# Autodesk Inventor assembly: 垃圾桶底座
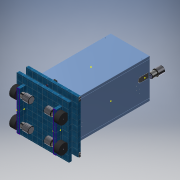
[picture p0: Inventor's stored thumbnail of the model, 180x180]
Saved by Autodesk Inventor 2017 (Build 210142000, 142)
## iProperties
Part Number: 垃圾桶底座
Material: 常规
Document SubType Name: Assembly
Designer: PANDA
Author: PANDA
## Documents named in this file (22)
- D:\PANDA\Study\VG100\P2\草图\垃圾桶丝轴滑杆\垃圾桶底座.iam
- D:\PANDA\Study\VG100\P2\草图\垃圾桶丝轴滑杆\垃圾桶正版.ipt
- D:\PANDA\Study\VG100\P2\草图\垃圾桶丝轴滑杆\垃圾桶侧板.ipt
- D:\PANDA\Study\VG100\P2\草图\垃圾桶丝轴滑杆\垃圾桶底板.ipt
- D:\PANDA\Study\VG100\P2\草图\垃圾桶丝轴滑杆\圆柱.ipt
- D:\PANDA\Study\VG100\P2\草图\垃圾桶丝轴滑杆\马达安装板.ipt
- D:\PANDA\Study\VG100\P2\草图\垃圾桶丝轴滑杆\轮子.ipt
- D:\PANDA\Study\VG100\P2\草图\垃圾桶丝轴滑杆\马达.ipt
- D:\PANDA\Study\VG100\P2\草图\垃圾桶丝轴滑杆\红外.ipt
- D:\PANDA\Study\VG100\P2\草图\垃圾桶丝轴滑杆\红外测距.ipt
- D:\PANDA\Study\VG100\P2\草图\垃圾桶丝轴滑杆\姿态传感器.ipt
- D:\PANDA\Study\VG100\P2\草图\垃圾桶丝轴滑杆\激光传感器.ipt
- D:\PANDA\Study\VG100\P2\草图\垃圾桶丝轴滑杆\内层升降板.ipt
- D:\PANDA\Study\VG100\P2\草图\垃圾桶丝轴滑杆\内层正板.ipt
- D:\PANDA\Study\VG100\P2\草图\垃圾桶丝轴滑杆\内层侧板.ipt
- D:\PANDA\Study\VG100\P2\草图\垃圾桶丝轴滑杆\推杆电机.ipt
- D:\PANDA\Study\VG100\P2\草图\垃圾桶丝轴滑杆\打包支架.ipt
- D:\PANDA\Study\VG100\P2\草图\垃圾桶丝轴滑杆\压缩杆.ipt
- D:\PANDA\Study\VG100\P2\草图\垃圾桶丝轴滑杆\滑竿固定器.ipt
- D:\PANDA\Study\VG100\P2\草图\垃圾桶丝轴滑杆\长轴.ipt
- D:\PANDA\Study\VG100\P2\草图\垃圾桶丝轴滑杆\丝杆.ipt
- D:\PANDA\Study\VG100\P2\草图\垃圾桶丝轴滑杆\升降板.ipt
## Components (59 placed, 21 different names)
1. 垃圾桶正版:1 — 旋转:3, 旋转:7, 旋转:8, 旋转:14
2. 垃圾桶侧板:2 — 旋转:3, 旋转:4, 旋转:5, 旋转:13, 刚性:22, 旋转:67, 旋转:68, 旋转:70, 旋转:81
3. 垃圾桶正版:2 — 旋转:4, 旋转:5, 旋转:6, 旋转:11
4. 垃圾桶侧板:3 — 旋转:6, 旋转:7, 旋转:12, 旋转:58, 旋转:63, 旋转:64, 旋转:65, 旋转:78
5. 垃圾桶底板:1 — 旋转:8, 旋转:9, 旋转:10, 旋转:15, 旋转:16, 刚性:2, 刚性:3, 刚性:4, 刚性:5, 刚性:21
6. 圆柱:1 — 旋转:9
7. 圆柱:2 — 旋转:10, 旋转:23
8. 圆柱:3 — 旋转:12, 旋转:19
9. 圆柱:4 — 旋转:11
10. 圆柱:5 — 旋转:15
11. 圆柱:6 — 旋转:16, 旋转:17, 旋转:18
12. 圆柱:7 — 旋转:14
13. 圆柱:8 — 旋转:13, 旋转:22
14. 垃圾桶底板:2 — 旋转:17, 刚性:1
15. 马达安装板:1 — 旋转:18, 旋转:19, 旋转:20, 旋转:21
16. 轮子:1 — 旋转:21, 旋转:29
17. 轮子:2 — 旋转:20, 旋转:28
18. 马达安装板:2 — 旋转:22, 旋转:23, 旋转:24, 旋转:25
19. 轮子:3 — 旋转:25, 旋转:27
20. 轮子:4 — 旋转:24, 旋转:26
21. 马达:1 — 旋转:26
22. 马达:2 — 旋转:27
23. 马达:3 — 旋转:28
24. 马达:4 — 旋转:29
25. 红外:1 — 刚性:1
26. 红外测距:1 — 刚性:2
27. 红外测距:2 — 刚性:3
28. 红外测距:3 — 刚性:5
29. 红外测距:4 — 刚性:4
30. 内层升降板:1 — 旋转:44, 旋转:45, 旋转:46, 旋转:47, 旋转:48
31. 内层正板:1 — 旋转:44, 旋转:57
32. 内层正板:2 — 旋转:45, 刚性:20
33. 内层侧板:1 — 旋转:46
34. 内层侧板:2 — 旋转:47, 旋转:48
35. 激光传感器:3 — 刚性:20
36. 激光传感器:4 — 旋转:57
37. 姿态传感器:1 — 刚性:21
38. 推杆电机:1 — 旋转:58, 旋转:60
39. 打包支架:1 — 旋转:59, 旋转:62
40. 打包支架:2 — 旋转:60, 旋转:61
41. 推杆电机:2 — 刚性:22, 旋转:59
42. 压缩杆:1 — 旋转:61
43. 压缩杆:2 — 旋转:62
44. 滑竿固定器:1 — 旋转:63, 刚性:23
45. 滑竿固定器:2 — 旋转:67, 旋转:77
46. 滑竿固定器:3 — 旋转:64
47. 滑竿固定器:4 — 旋转:65
48. 滑竿固定器:6 — 旋转:70
49. 滑竿固定器:8 — 旋转:68
50. 丝杆:1 — 旋转:77, 刚性:24
51. 丝杆:2 — 刚性:23, 旋转:85
52. 滑竿固定器:9 — 旋转:78, 旋转:80
53. 长轴:1 — 旋转:80, 旋转:84
54. 马达:5 — 旋转:83
55. 马达:6 — 旋转:84
56. 滑竿固定器:10 — 旋转:81, 旋转:82
57. 长轴:2 — 旋转:82, 旋转:83
58. 升降板:2 — 刚性:24
59. 升降板:3 — 旋转:85
## Relationships (62: RevoluteJoint 52, WeldJoint 10)
- 旋转:3 [RevoluteJoint]: 垃圾桶正版:1 ↔ 垃圾桶侧板:2
- 旋转:4 [RevoluteJoint]: 垃圾桶侧板:2 ↔ 垃圾桶正版:2
- 旋转:5 [RevoluteJoint]: 垃圾桶侧板:2 ↔ 垃圾桶正版:2
- 旋转:6 [RevoluteJoint]: 垃圾桶正版:2 ↔ 垃圾桶侧板:3
- 旋转:7 [RevoluteJoint]: 垃圾桶正版:1 ↔ 垃圾桶侧板:3
- 旋转:8 [RevoluteJoint]: 垃圾桶正版:1 ↔ 垃圾桶底板:1
- 旋转:9 [RevoluteJoint]: 垃圾桶底板:1 ↔ 圆柱:1
- 旋转:10 [RevoluteJoint]: 垃圾桶底板:1 ↔ 圆柱:2
- 旋转:11 [RevoluteJoint]: 垃圾桶正版:2 ↔ 圆柱:4
- 旋转:12 [RevoluteJoint]: 垃圾桶侧板:3 ↔ 圆柱:3
- 旋转:13 [RevoluteJoint]: 垃圾桶侧板:2 ↔ 圆柱:8
- 旋转:14 [RevoluteJoint]: 垃圾桶正版:1 ↔ 圆柱:7
- 旋转:15 [RevoluteJoint]: 垃圾桶底板:1 ↔ 圆柱:5
- 旋转:16 [RevoluteJoint]: 垃圾桶底板:1 ↔ 圆柱:6
- 旋转:17 [RevoluteJoint]: 圆柱:6 ↔ 垃圾桶底板:2
- 旋转:18 [RevoluteJoint]: 圆柱:6 ↔ 马达安装板:1
- 旋转:19 [RevoluteJoint]: 圆柱:3 ↔ 马达安装板:1
- 旋转:20 [RevoluteJoint]: 马达安装板:1 ↔ 轮子:2
- 旋转:21 [RevoluteJoint]: 马达安装板:1 ↔ 轮子:1
- 旋转:22 [RevoluteJoint]: 圆柱:8 ↔ 马达安装板:2
- 旋转:23 [RevoluteJoint]: 圆柱:2 ↔ 马达安装板:2
- 旋转:24 [RevoluteJoint]: 马达安装板:2 ↔ 轮子:4
- 旋转:25 [RevoluteJoint]: 马达安装板:2 ↔ 轮子:3
- 旋转:26 [RevoluteJoint]: 轮子:4 ↔ 马达:1
- 旋转:27 [RevoluteJoint]: 轮子:3 ↔ 马达:2
- 旋转:28 [RevoluteJoint]: 轮子:2 ↔ 马达:3
- 旋转:29 [RevoluteJoint]: 轮子:1 ↔ 马达:4
- 刚性:1 [WeldJoint]: 垃圾桶底板:2 ↔ 红外:1
- 刚性:2 [WeldJoint]: 垃圾桶底板:1 ↔ 红外测距:1
- 刚性:3 [WeldJoint]: 垃圾桶底板:1 ↔ 红外测距:2
- 刚性:4 [WeldJoint]: 垃圾桶底板:1 ↔ 红外测距:4
- 刚性:5 [WeldJoint]: 垃圾桶底板:1 ↔ 红外测距:3
- 旋转:44 [RevoluteJoint]: 内层升降板:1 ↔ 内层正板:1
- 旋转:45 [RevoluteJoint]: 内层升降板:1 ↔ 内层正板:2
- 旋转:46 [RevoluteJoint]: 内层升降板:1 ↔ 内层侧板:1
- 旋转:47 [RevoluteJoint]: 内层升降板:1 ↔ 内层侧板:2
- 旋转:48 [RevoluteJoint]: 内层升降板:1 ↔ 内层侧板:2
- 刚性:20 [WeldJoint]: 内层正板:2 ↔ 激光传感器:3
- 旋转:57 [RevoluteJoint]: 内层正板:1 ↔ 激光传感器:4
- 刚性:21 [WeldJoint]: 垃圾桶底板:1 ↔ 姿态传感器:1
- 旋转:58 [RevoluteJoint]: 垃圾桶侧板:3 ↔ 推杆电机:1
- 刚性:22 [WeldJoint]: 垃圾桶侧板:2 ↔ 推杆电机:2
- 旋转:59 [RevoluteJoint]: 打包支架:1 ↔ 推杆电机:2
- 旋转:60 [RevoluteJoint]: 推杆电机:1 ↔ 打包支架:2
- 旋转:61 [RevoluteJoint]: 打包支架:2 ↔ 压缩杆:1
- 旋转:62 [RevoluteJoint]: 打包支架:1 ↔ 压缩杆:2
- 旋转:63 [RevoluteJoint]: 垃圾桶侧板:3 ↔ 滑竿固定器:1
- 旋转:64 [RevoluteJoint]: 垃圾桶侧板:3 ↔ 滑竿固定器:3
- 旋转:65 [RevoluteJoint]: 垃圾桶侧板:3 ↔ 滑竿固定器:4
- 旋转:67 [RevoluteJoint]: 垃圾桶侧板:2 ↔ 滑竿固定器:2
- 旋转:68 [RevoluteJoint]: 垃圾桶侧板:2 ↔ 滑竿固定器:8
- 旋转:70 [RevoluteJoint]: 垃圾桶侧板:2 ↔ 滑竿固定器:6
- 旋转:77 [RevoluteJoint]: 滑竿固定器:2 ↔ 丝杆:1
- 刚性:23 [WeldJoint]: 滑竿固定器:1 ↔ 丝杆:2
- 旋转:78 [RevoluteJoint]: 垃圾桶侧板:3 ↔ 滑竿固定器:9
- 旋转:80 [RevoluteJoint]: 滑竿固定器:9 ↔ 长轴:1
- 旋转:81 [RevoluteJoint]: 垃圾桶侧板:2 ↔ 滑竿固定器:10
- 旋转:82 [RevoluteJoint]: 滑竿固定器:10 ↔ 长轴:2
- 旋转:83 [RevoluteJoint]: 马达:5 ↔ 长轴:2
- 旋转:84 [RevoluteJoint]: 长轴:1 ↔ 马达:6
- 刚性:24 [WeldJoint]: 丝杆:1 ↔ 升降板:2
- 旋转:85 [RevoluteJoint]: 丝杆:2 ↔ 升降板:3
